# Autodesk Inventor assembly: Camera
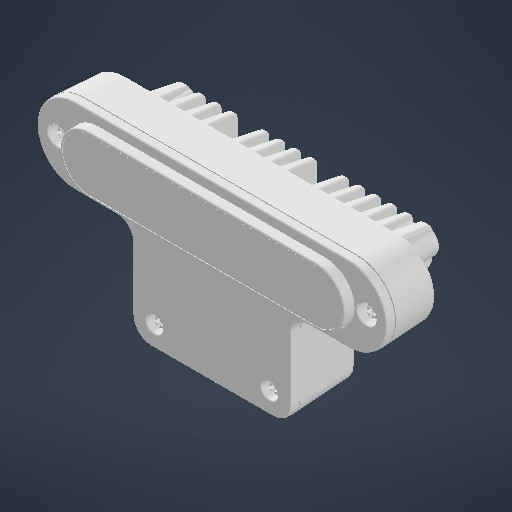
[picture p0: Inventor's stored thumbnail of the model, 512x512]
Saved by Autodesk Inventor 2026.2 (Build 302298000, 298)
## iProperties
Created: 2022-01-14
Part Number: Camera
Document SubType Name: Assembly
Designer: User
Sending System: CREO PARAMETRIC BY PTC INC, 2020154
Preprocessor: CREO PARAMETRIC BY PTC INC, 2020154
Title: 010-00002_ASM
Author: TWSung
Revision Number: 4LAST_VERSION
## Documents named in this file (8)
- C:\Users\User\Documents\4TB6 - Capstone\Code Git\PlantMama\rev_0\Camera.iam
- C:\Users\User\Downloads\BW1098OAK_enclosure\BW1098OAK_enclosure\606-00007.ipt
- C:\Users\User\Downloads\BW1098OAK_enclosure\BW1098OAK_enclosure\605-00001.ipt
- C:\Users\User\Downloads\BW1098OAK_enclosure\BW1098OAK_enclosure\602-00002.ipt
- C:\Users\User\Downloads\BW1098OAK_enclosure\BW1098OAK_enclosure\609-00002_ASM.iam
- C:\Users\User\Downloads\BW1098OAK_enclosure\BW1098OAK_enclosure\611-00002.ipt
- C:\Users\User\Downloads\BW1098OAK_enclosure\BW1098OAK_enclosure\611-00014.ipt
- C:\Users\User\Downloads\BW1098OAK_enclosure\BW1098OAK_enclosure\611-00005.ipt
## Components (16 placed, 16 different names)
1. 606-00007_0 — Symmetry:1
2. 605-00001_1
3. 602-00002_2
4. 602-00002_3
5. 602-00002_4
6. 602-00002_5
7. 609-00002_ASM_8 [sub-assembly]
8. 611-00002_9
9. 611-00002_10
10. 602-00002_11
11. 602-00002_12
12. 602-00002_13
13. 602-00002_14
14. 611-00014_15
15. 611-00005_16 — Symmetry:1
16. 611-00005_17
## Relationships (1: Symmetry 1)
- Symmetry:1: 606-00007_0 ↔ 611-00005_16
